# Autodesk Inventor assembly: Ensemble tout
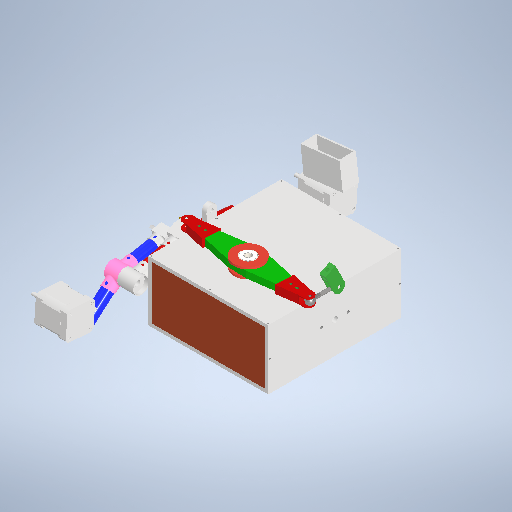
[picture p0: Inventor's stored thumbnail of the model, 512x512]
Saved by Autodesk Inventor 2026.2 (Build 302298010, 298A)
## iProperties
Created: 2026-03-16
Part Number: Ensemble tout
Document SubType Name: Assembly
Designer: genon
Author: genon
## Documents named in this file (7)
- C:\Users\genon\Documents\Henallux Passerelle\Projet de conception\Cassini T-X\Inventor\Ensemble tout.iam
- C:\Users\genon\Documents\Henallux Passerelle\Projet de conception\Cassini T-X\Inventor\Ensemble_Boite_chassis.iam
- C:\Users\genon\Documents\Henallux Passerelle\Projet de conception\Cassini T-X\Inventor\Suspension\Ensemble_Relier_suspension.iam
- C:\Users\genon\Documents\Henallux Passerelle\Projet de conception\Cassini T-X\Inventor\Suspension\Ensemble côté suspension.iam
- C:\Users\genon\Documents\Henallux Passerelle\Projet de conception\Cassini T-X\Inventor\Suspension\tube vers bogie.ipt
- C:\Users\genon\Documents\Inventor\Content Center Files\R2025\fr-FR\DIN 444\DIN 444 - A - M5 x 30 5.ipt
- C:\Users\genon\Documents\Henallux Passerelle\Projet de conception\Cassini T-X\Inventor\Suspension\bielle sup.ipt
## Components (6 placed, 6 different names)
1. Ensemble_Boite_chassis:1 [sub-assembly] — Placage:1, Placage:2, Placage:6, Placage:7, Placage:8
2. Ensemble_Relier_suspension:1 [sub-assembly] — Placage:1, Placage:2, Cylindrique:1
3. Ensemble côté suspension:2 [sub-assembly] — Placage:6, Placage:7, Placage:8, Placage:13, Placage:14
4. tube vers bogie:2 — Placage:13, Placage:14
5. DIN 444 A - M5 x 30:1 — Cylindrique:1
6. bielle sup:1
## Relationships (8: Mate 7, CylindricalJoint 1)
- Placage:1 [Mate]: Ensemble_Boite_chassis:1 ↔ Ensemble_Relier_suspension:1
- Placage:2 [Mate]: Ensemble_Boite_chassis:1 ↔ Ensemble_Relier_suspension:1
- Placage:6 [Mate]: Ensemble_Boite_chassis:1 ↔ Ensemble côté suspension:2
- Placage:7 [Mate]: Ensemble_Boite_chassis:1 ↔ Ensemble côté suspension:2
- Placage:8 [Mate]: Ensemble_Boite_chassis:1 ↔ Ensemble côté suspension:2
- Placage:13 [Mate]: Ensemble côté suspension:2 ↔ tube vers bogie:2
- Placage:14 [Mate]: Ensemble côté suspension:2 ↔ tube vers bogie:2
- Cylindrique:1: Ensemble_Relier_suspension:1 ↔ DIN 444 A - M5 x 30:1
